# Autodesk Inventor assembly: Hitbox
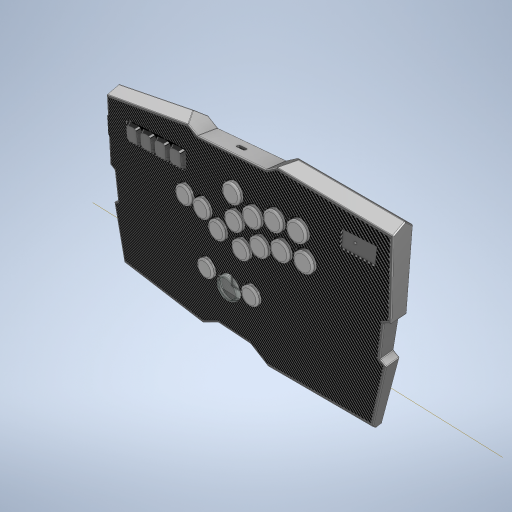
[picture p0: Inventor's stored thumbnail of the model, 512x512]
Saved by Autodesk Inventor 2024 (Build 280153000, 153)
## iProperties
Created: 2023-09-15
Part Number: Hitbox
Document SubType Name: Assembly
Designer: nicx5
Author: nicx5
## Documents named in this file (8)
- E:\Works\Hitbox_CNC\Hitbox.iam
- E:\Works\Hitbox_CNC\Bottom_Plate.ipt
- E:\Works\Hitbox_CNC\Frame.ipt
- E:\Works\Hitbox_CNC\Positioning_Plate.ipt
- E:\Works\Hitbox_CNC\Top_Plate.ipt
- E:\Works\Hitbox_CNC\Buttonx20.ipt
- E:\Works\Hitbox_CNC\Buttonx26.ipt
- E:\Works\Hitbox_CNC\Button_16x16.ipt
## Components (23 placed, 7 different names)
1. Bottom_Plate:1 — 配合:36
2. Frame:1 — 配合:34, 配合:35, 配合:36, 配合:37, 配合:38, 配合:39
3. Positioning_Plate:1 — 配合:34, 配合:35
4. Top_Plate:1 — 配合:37, 配合:38, 配合:39
5. Buttonx20:1
6. Buttonx20:2
7. Buttonx20:3
8. Buttonx20:4
9. Buttonx20:5
10. Buttonx20:6
11. Buttonx20:7
12. Buttonx20:8
13. Buttonx20:9
14. Buttonx20:10
15. Buttonx20:11
16. Buttonx20:12
17. Buttonx20:13
18. Buttonx20:14
19. Buttonx26:1
20. Button_16x16:1
21. Button_16x16:2
22. Button_16x16:3
23. Button_16x16:4
## Relationships (6: Mate 6)
- 配合:34 [Mate]: Frame:1 ↔ Positioning_Plate:1
- 配合:35 [Mate]: Frame:1 ↔ Positioning_Plate:1
- 配合:36 [Mate]: Bottom_Plate:1 ↔ Frame:1
- 配合:37 [Mate]: Frame:1 ↔ Top_Plate:1
- 配合:38 [Mate]: Frame:1 ↔ Top_Plate:1
- 配合:39 [Mate]: Frame:1 ↔ Top_Plate:1
